# Autodesk Inventor assembly: Rb PEEK
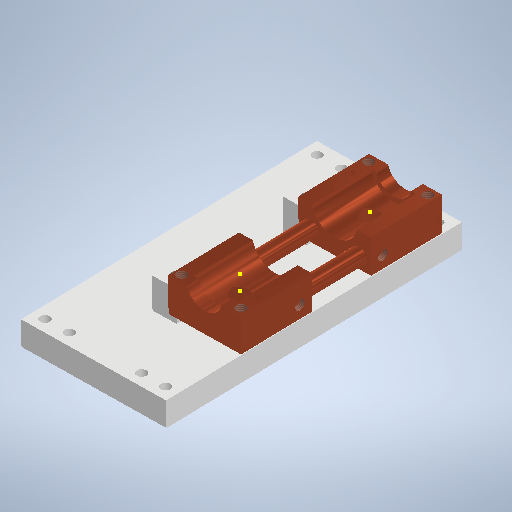
[picture p0: Inventor's stored thumbnail of the model, 512x512]
Saved by Autodesk Inventor 2025.3 (Build 293356000, 356)
## iProperties
Created: 2025-05-09
Part Number: Rb PEEK
Document SubType Name: Assembly
Designer: E. Moreno
Author: E. Moreno
Title: Rb PEEK - Ensamblado
## Documents named in this file (8)
- E:\Users\USER\Documents\GitHub\LAFriOC\Rb oven\Rb Full.iam
- E:\Users\USER\Documents\GitHub\LAFriOC\Rb oven\Rb PEEK\Rb PEEK - Arriba.ipt
- E:\Users\USER\Documents\GitHub\LAFriOC\Rb oven\Rb PEEK\Rb PEEK - Largo.ipt
- E:\Users\USER\Documents\GitHub\LAFriOC\Rb oven\Rb PEEK\Rb PEEK - Corto con ventana.ipt
- E:\Users\USER\Documents\GitHub\LAFriOC\Rb oven\Rb PEEK\Rb PEEK - Largo_MIR.ipt
- E:\Users\USER\Documents\GitHub\LAFriOC\Rb oven\Rb PEEK\Rb PEEK - Soporte.ipt
- E:\Users\USER\Documents\GitHub\LAFriOC\Rb oven\Rb PEEK\Rb PEEK - Abajo.ipt
- E:\Users\USER\Documents\GitHub\LAFriOC\Rb oven\Rb oven housing\Rb oven housing - Bottom.iam
## Components (9 placed, 7 different names)
1. Rb PEEK - Arriba:1 — Mate:1, Mate:2, Mate:3, Mate:5, Mate:6, Mate:11, Mate:12
2. Rb PEEK - Largo:1 — Mate:1, Mate:2, Mate:3, Mate:4, Mate:18, Mate:20, Mate:21, Mate:22, Mate:23
3. Rb PEEK - Corto con ventana:1 — Mate:4, Mate:5, Mate:6
4. Rb PEEK - Largo_MIR:1 — Mate:11, Mate:12, Mate:26, Mate:27, Mate:28
5. Rb PEEK - Soporte:1 — Mate:25
6. Rb PEEK - Soporte:2 — Mate:24, Mate:29
7. Rb PEEK - Corto con ventana:2 — Mate:18, Mate:20
8. Rb PEEK - Abajo:1 — Mate:21, Mate:22, Mate:23, Mate:24, Mate:25, Mate:26, Mate:27, Mate:28
9. Rb oven housing - Bottom:1 [sub-assembly] — Mate:29
## Relationships (19: Mate 19)
- Mate:1: Rb PEEK - Arriba:1 ↔ Rb PEEK - Largo:1
- Mate:2: Rb PEEK - Arriba:1 ↔ Rb PEEK - Largo:1
- Mate:3: Rb PEEK - Arriba:1 ↔ Rb PEEK - Largo:1
- Mate:4: Rb PEEK - Largo:1 ↔ Rb PEEK - Corto con ventana:1
- Mate:5: Rb PEEK - Arriba:1 ↔ Rb PEEK - Corto con ventana:1
- Mate:6: Rb PEEK - Arriba:1 ↔ Rb PEEK - Corto con ventana:1
- Mate:11: Rb PEEK - Arriba:1 ↔ Rb PEEK - Largo_MIR:1
- Mate:12: Rb PEEK - Arriba:1 ↔ Rb PEEK - Largo_MIR:1
- Mate:18: Rb PEEK - Largo:1 ↔ Rb PEEK - Corto con ventana:2
- Mate:20: Rb PEEK - Largo:1 ↔ Rb PEEK - Corto con ventana:2
- Mate:21: Rb PEEK - Largo:1 ↔ Rb PEEK - Abajo:1
- Mate:22: Rb PEEK - Largo:1 ↔ Rb PEEK - Abajo:1
- Mate:23: Rb PEEK - Largo:1 ↔ Rb PEEK - Abajo:1
- Mate:24: Rb PEEK - Soporte:2 ↔ Rb PEEK - Abajo:1
- Mate:25: Rb PEEK - Soporte:1 ↔ Rb PEEK - Abajo:1
- Mate:26: Rb PEEK - Largo_MIR:1 ↔ Rb PEEK - Abajo:1
- Mate:27: Rb PEEK - Largo_MIR:1 ↔ Rb PEEK - Abajo:1
- Mate:28: Rb PEEK - Largo_MIR:1 ↔ Rb PEEK - Abajo:1
- Mate:29: Rb PEEK - Soporte:2 ↔ Rb oven housing - Bottom:1
